# Autodesk Inventor assembly: sb_lid_assembly
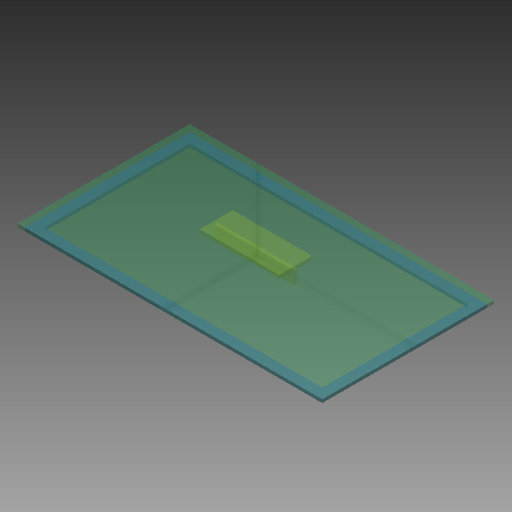
[picture p0: Inventor's stored thumbnail of the model, 512x512]
Saved by Autodesk Inventor 2018.1 (Build 221171000, 171)
## iProperties
Created: 2017-08-17
Part Number: sb_lid_assembly
Document SubType Name: Assembly
Designer: Tom
Author: Tom
## Documents named in this file (5)
- \\Mac\Dropbox\2015-2016\Bachelorproef\Inventor\Electronics and Solenoids Box\eb_lid_assembly.iam
- \\Mac\Dropbox\2015-2016\Bachelorproef\Inventor\Electronics and Solenoids Box\eb_top.ipt
- \\Mac\Dropbox\2015-2016\Bachelorproef\Inventor\Electronics and Solenoids Box\tank_lid_handle_assembly.iam
- \\Mac\Dropbox\2015-2016\Bachelorproef\Inventor\Electronics and Solenoids Box\eb_top_support.ipt
- \\Mac\Dropbox\2015-2016\Bachelorproef\Inventor\Electronics and Solenoids Box\par_sol_box.xls
## Components (3 placed, 3 different names)
1. eb_top:1 — Mate:12, Flush:10, Flush:11, Mate:13, Flush:12, Flush:13
2. tank_lid_handle_assembly:2 [sub-assembly] — Mate:12, Flush:10, Flush:11
3. eb_top_support:1 — Mate:13, Flush:12, Flush:13
## Relationships (6: Flush 4, Mate 2)
- Mate:12: eb_top:1 ↔ tank_lid_handle_assembly:2
- Flush:10 (127.5 mm): eb_top:1 ↔ tank_lid_handle_assembly:2
- Flush:11 (170 mm): eb_top:1 ↔ tank_lid_handle_assembly:2
- Mate:13: eb_top:1 ↔ eb_top_support:1
- Flush:12 (-5.5 mm): eb_top:1 ↔ eb_top_support:1
- Flush:13 (5.5 mm): eb_top:1 ↔ eb_top_support:1
## Named parameters: solhole = 3 mm, solholespacing = 16 mm, ssoll = 70 mm, ssolw = 63 mm, bsoll = 126 mm, bsolw = 91 mm, bsolh = 126 mm, tapl = 31 mm, tl = 32 mm, tw = 50 mm, eloboww = 25 mm, pvct = 5 mm, boxw = 450 mm, boxl = 250 mm, boxh = 258 mm, supporth = 15 mm, play = 0.5 mm, sidedist = 90 mm, pcbw = 76 mm, pcbh = 46 mm, psul = 140 mm, screenl = 115 mm, screent = 50 mm, psuw = 150 mm, pcbl = 86 mm, arl = 102 mm, psuh = 85 mm, arw = 54 mm, screenw = 197 mm, seph = 105 mm, diapower = 16 mm, diaphouter = 48 mm, diaph = 32 mm, diapowerouter = 25 mm, diaload = 16 mm, diaetape = 25 mm, diaetapeouter = 36 mm, dialoadouter = 25 mm, airoutinner = 28 mm, waterinner = 28 mm, distpumps = 75 mm, distsidepump = 120 mm, waterouter = 39 mm, pumpinner = 16 mm, pumpouter = 25 mm, distbubblewater = 82 mm, distpumpbubble = 100 mm, airinouter = 39 mm, airoutouter = 39 mm, airininner = 28 mm, distsidewater = 100 mm
